# Autodesk Inventor assembly: Bedienhebel
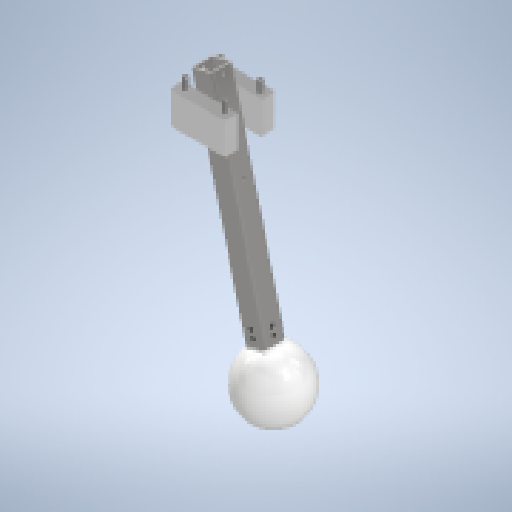
[picture p0: Inventor's stored thumbnail of the model, 512x512]
Saved by Autodesk Inventor 2025 (Build 290162010, 162A)
## iProperties
Created: 2024-11-27
Part Number: Bedienhebel
Document SubType Name: Assembly
Designer: Admin
Author: Admin
## Documents named in this file (9)
- C:\Users\Admin\Documents\Inventor\Krandemonstrator\Bedienhebel.iam
- C:\Users\Admin\Documents\Inventor\Krandemonstrator\HebelhalterBlock.ipt
- C:\Users\Admin\Documents\Inventor\Krandemonstrator\HebelhalterBlockBlind.ipt
- C:\Users\Admin\Documents\Inventor\Krandemonstrator\ISO 12633-2 - 20x20x2 - 200.ipt
- C:\Users\Admin\Documents\Inventor\Krandemonstrator\knauf.ipt
- C:\Users\Admin\Documents\Inventor\Content Center Files\R2025\de-DE\ISO 1482 - C(1)\DIN EN ISO 1482 - ST2,2 x 6,5_ - C.ipt
- C:\Users\Admin\Documents\Inventor\Content Center Files\R2025\de-DE\DIN 7991(2)\DIN 7991 - M4x40.ipt
- C:\Users\Admin\Documents\Inventor\Content Center Files\R2025\de-DE\AS 1237 (2.1)\AS 1237 - 4.ipt
- C:\Users\Admin\Documents\Inventor\Krandemonstrator\Lagerhülse 6x4x0.ipt
## Components (20 placed, 8 different names)
1. HebelhalterBlock:1 — Passend:1, Passend:2, Passend:5, Starr:3, Drehbar:1, Starr:5
2. HebelhalterBlockBlind:1 — Passend:3, Passend:4, Starr:4, Starr:5
3. DIN 7991 M4x40:2 — Passend:1
4. DIN 7991 M4x40:3 — Passend:2
5. DIN 7991 M4x40:4 — Passend:3
6. DIN 7991 M4x40:5 — Passend:4
7. DIN 7991 M4x40:1 — Passend:5
8. ISO 12633-2 - 20x20x2 - 200:1 — Starr:1, Passend:6, Passend:7, Passend:8, Passend:9, Passend:10, Passend:11, Passend:12, Passend:13, Drehbar:1, Drehbar:2
9. knauf:1 — Starr:1
10. DIN EN ISO 1482 - C ST2,2 x 6,5 - C:1 — Passend:6
11. DIN EN ISO 1482 - C ST2,2 x 6,5 - C:2 — Passend:7
12. DIN EN ISO 1482 - C ST2,2 x 6,5 - C:3 — Passend:8
13. DIN EN ISO 1482 - C ST2,2 x 6,5 - C:4 — Passend:9
14. DIN EN ISO 1482 - C ST2,2 x 6,5 - C:5 — Passend:10
15. DIN EN ISO 1482 - C ST2,2 x 6,5 - C:6 — Passend:11
16. DIN EN ISO 1482 - C ST2,2 x 6,5 - C:7 — Passend:12
17. DIN EN ISO 1482 - C ST2,2 x 6,5 - C:8 — Passend:13
18. AS 1237 (2.1) 4:1 — Starr:4
19. AS 1237 (2.1) 4:2 — Starr:3
20. Lagerhülse 6x4x0:1 — Drehbar:2
## Relationships (19: Mate 13, WeldJoint 4, RevoluteJoint 2)
- Passend:1 [Mate]: HebelhalterBlock:1 ↔ DIN 7991 M4x40:2
- Passend:2 [Mate]: HebelhalterBlock:1 ↔ DIN 7991 M4x40:3
- Passend:3 [Mate]: HebelhalterBlockBlind:1 ↔ DIN 7991 M4x40:4
- Passend:4 [Mate]: HebelhalterBlockBlind:1 ↔ DIN 7991 M4x40:5
- Passend:5 [Mate]: HebelhalterBlock:1 ↔ DIN 7991 M4x40:1
- Starr:1 [WeldJoint]: ISO 12633-2 - 20x20x2 - 200:1 ↔ knauf:1
- Passend:6 [Mate]: ISO 12633-2 - 20x20x2 - 200:1 ↔ DIN EN ISO 1482 - C ST2,2 x 6,5 - C:1
- Passend:7 [Mate]: ISO 12633-2 - 20x20x2 - 200:1 ↔ DIN EN ISO 1482 - C ST2,2 x 6,5 - C:2
- Passend:8 [Mate]: ISO 12633-2 - 20x20x2 - 200:1 ↔ DIN EN ISO 1482 - C ST2,2 x 6,5 - C:3
- Passend:9 [Mate]: ISO 12633-2 - 20x20x2 - 200:1 ↔ DIN EN ISO 1482 - C ST2,2 x 6,5 - C:4
- Passend:10 [Mate]: ISO 12633-2 - 20x20x2 - 200:1 ↔ DIN EN ISO 1482 - C ST2,2 x 6,5 - C:5
- Passend:11 [Mate]: ISO 12633-2 - 20x20x2 - 200:1 ↔ DIN EN ISO 1482 - C ST2,2 x 6,5 - C:6
- Passend:12 [Mate]: ISO 12633-2 - 20x20x2 - 200:1 ↔ DIN EN ISO 1482 - C ST2,2 x 6,5 - C:7
- Passend:13 [Mate]: ISO 12633-2 - 20x20x2 - 200:1 ↔ DIN EN ISO 1482 - C ST2,2 x 6,5 - C:8
- Starr:3 [WeldJoint]: HebelhalterBlock:1 ↔ AS 1237 (2.1) 4:2
- Drehbar:1 [RevoluteJoint] (1 mm): HebelhalterBlock:1 ↔ ISO 12633-2 - 20x20x2 - 200:1
- Starr:4 [WeldJoint]: HebelhalterBlockBlind:1 ↔ AS 1237 (2.1) 4:1
- Starr:5 [WeldJoint] (-22 mm): HebelhalterBlock:1 ↔ HebelhalterBlockBlind:1
- Drehbar:2 [RevoluteJoint]: ISO 12633-2 - 20x20x2 - 200:1 ↔ Lagerhülse 6x4x0:1
